# Autodesk Inventor assembly: osszekotoelem
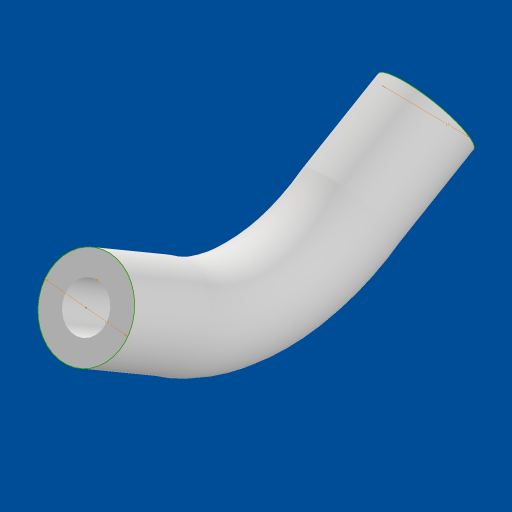
[picture p0: Inventor's stored thumbnail of the model, 512x512]
Saved by Autodesk Inventor 2023 (Build 270158000, 158)
## iProperties
Created: 2022-11-21
Part Number: osszekotoelem
Document SubType Name: Assembly
Designer: gd1
Author: gd1
## Documents named in this file (2)
- C:\Users\gd1\3D Objects\3D nagyteherbírású híd\Híd\H-d\osszekotoelem.iam
- C:\Users\gd1\3D Objects\3D nagyteherbírású híd\Híd\H-d\OSSZEKOTOELEM.ipt
## Components (1 placed, 1 different names)
1. OSSZEKOTOELEM:1 — Mate:1, Angle:1, Mate:2, Angle:2
## Relationships (4: Mate 2, Angle 2)
- Mate:1: OSSZEKOTOELEM:1
- Angle:1 (0 deg): OSSZEKOTOELEM:1
- Mate:2: OSSZEKOTOELEM:1
- Angle:2 (0 deg): OSSZEKOTOELEM:1
